# Autodesk Inventor assembly: T2601_EG
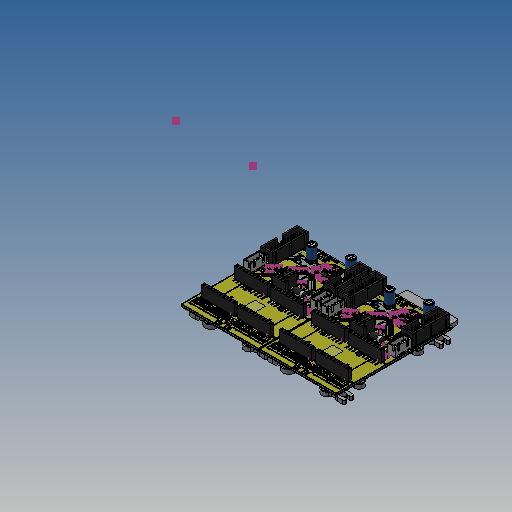
[picture p0: Inventor's stored thumbnail of the model, 512x512]
Saved by Autodesk Inventor 2025.3 (Build 293356000, 356)
## iProperties
Created: 2026-09-18
Part Number: T2601_EG
Project: Nom Projet
Description: Ens. Nom Ensemble
Document SubType Name: Assembly
Designer: jules
Mass: 0.0417569 g
Surface Area: 975.72 cm^2
Volume: 41.7569 cm^3
Density: 0.001 g/cm^3
Author: jules
## Documents named in this file (5)
- C:\Users\jules\OneDrive\PCB_Perso\T2601_APIArduino\T2601_Mecanique\T2601_EG.iam
- C:\Users\jules\OneDrive\PCB_Perso\T2601_APIArduino\T2601_Mecanique\T2601_ExtentionBoard\T2601_ExtentionBoard\T2601_ExtentionBoard.iam
- C:\Users\jules\OneDrive\PCB_Perso\T2601_APIArduino\T2601_Mecanique\T2601_BaseP30.ipt
- C:\Users\jules\OneDrive\PCB_Perso\T2601_APIArduino\T2601_Mecanique\T2601_Conn.ipt
- C:\Users\jules\OneDrive\PCB_Perso\T2601_APIArduino\T2601_Mecanique\T2601_SupportEtiq.ipt
## Components (7 placed, 4 different names)
1. T2601_ExtentionBoard:1 [sub-assembly] — Placage:1, Placage:2, Placage:3
2. T2601_BaseP30:1 — Placage:1, Placage:2, Placage:3, Affleurement:1, Placage:4, Affleurement:2, Angle:1, Placage:7, Affleurement:5
3. T2601_Conn:1 — Placage:6, Placage:7, Affleurement:4
4. T2601_Conn:2 — Placage:4, Placage:5, Affleurement:2, Affleurement:3
5. T2601_BaseP30:2 — Affleurement:1, Placage:5, Affleurement:3, Angle:1, Placage:6, Affleurement:4, Affleurement:5, Placage:8, Placage:9, Placage:10, Placage:11, Placage:12, Affleurement:6
6. T2601_ExtentionBoard:2 [sub-assembly] — Placage:8, Placage:9, Placage:10
7. T2601_SupportEtiq:1 — Placage:11, Placage:12, Affleurement:6
## Relationships (19: Mate 12, Flush 6, Angle 1)
- Placage:1 [Mate]: T2601_ExtentionBoard:1 ↔ T2601_BaseP30:1
- Placage:2 [Mate]: T2601_ExtentionBoard:1 ↔ T2601_BaseP30:1
- Placage:3 [Mate]: T2601_ExtentionBoard:1 ↔ T2601_BaseP30:1
- Affleurement:1 [Flush]: T2601_BaseP30:1 ↔ T2601_BaseP30:2
- Placage:4 [Mate]: T2601_BaseP30:1 ↔ T2601_Conn:2
- Placage:5 [Mate]: T2601_Conn:2 ↔ T2601_BaseP30:2
- Affleurement:2 [Flush]: T2601_BaseP30:1 ↔ T2601_Conn:2
- Affleurement:3 [Flush]: T2601_Conn:2 ↔ T2601_BaseP30:2
- Angle:1 (0 deg): T2601_BaseP30:1 ↔ T2601_BaseP30:2
- Placage:6 [Mate]: T2601_Conn:1 ↔ T2601_BaseP30:2
- Placage:7 [Mate]: T2601_BaseP30:1 ↔ T2601_Conn:1
- Affleurement:4 [Flush]: T2601_Conn:1 ↔ T2601_BaseP30:2
- Affleurement:5 [Flush]: T2601_BaseP30:1 ↔ T2601_BaseP30:2
- Placage:8 [Mate]: T2601_BaseP30:2 ↔ T2601_ExtentionBoard:2
- Placage:9 [Mate]: T2601_BaseP30:2 ↔ T2601_ExtentionBoard:2
- Placage:10 [Mate]: T2601_BaseP30:2 ↔ T2601_ExtentionBoard:2
- Placage:11 [Mate]: T2601_BaseP30:2 ↔ T2601_SupportEtiq:1
- Placage:12 [Mate]: T2601_BaseP30:2 ↔ T2601_SupportEtiq:1
- Affleurement:6 [Flush]: T2601_BaseP30:2 ↔ T2601_SupportEtiq:1
